# Autodesk Inventor assembly: 部件1
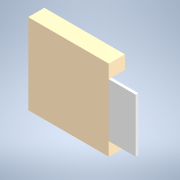
[picture p0: Inventor's stored thumbnail of the model, 180x180]
Saved by Autodesk Inventor 2020 (Build 240168000, 168)
## iProperties
Created: 2021-04-04
Part Number: 部件1
Document SubType Name: Weldment
Designer: 70929
Weld Material: Welded Aluminum-6061
Author: 70929
## Documents named in this file (4)
- D:\大创\图书整理机器人\建模\部件\部件1.iam
- D:\大创\图书整理机器人\建模\放书的.ipt
- D:\大创\图书整理机器人\建模\书.ipt
- D:\大创\图书整理机器人\建模\外置架.ipt
## Components (3 placed, 3 different names)
1. 放书的:2 — 角度:1, 配合:1, 配合:2, 刚性:1
2. 书:1 — 角度:1, 配合:1, 配合:2
3. 外置架:1 — 刚性:1
## Relationships (4: Mate 2, Angle 1, WeldJoint 1)
- 角度:1 [Angle] (0 deg): 放书的:2 ↔ 书:1
- 配合:1 [Mate]: 放书的:2 ↔ 书:1
- 配合:2 [Mate]: 放书的:2 ↔ 书:1
- 刚性:1 [WeldJoint]: 放书的:2 ↔ 外置架:1
